# Autodesk Inventor assembly: BoronProbe_5
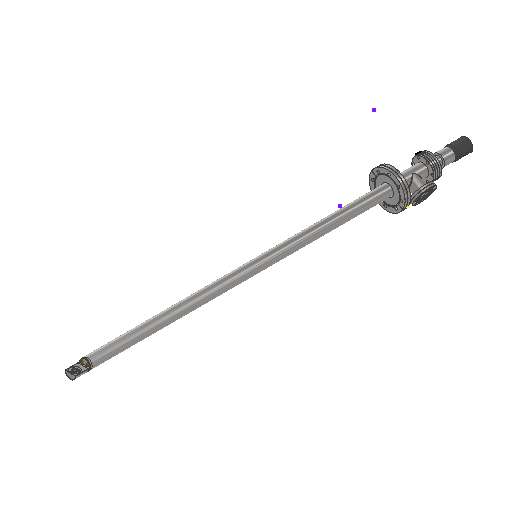
[picture p0: Inventor's stored thumbnail of the model, 512x512]
Saved by Autodesk Inventor 2026.2 (Build 302298000, 298)
## iProperties
Created: 2026-05-08
Part Number: BoronProbe_5
Document SubType Name: Assembly
Designer: zetsu
Author: zetsu
## Documents named in this file (22)
- D:\repos\PIHTI\BoronProbe_5\BoronProbe_5.iam
- D:\repos\PIHTI\BoronProbe_5\parts\B_probehead_5.ipt
- D:\repos\PIHTI\BoronProbe_5\parts\B_holder_sub_5.ipt
- D:\repos\PIHTI\BoronProbe_5\parts\B_pipe_cylinder_5.ipt
- D:\repos\PIHTI\BoronProbe_5\parts\M3x6-BHCS.ipt
- D:\repos\PIHTI\BoronProbe_5\parts\ceramic_bushing_M3-v1.ipt
- D:\repos\PIHTI\BoronProbe_5\parts\ceramic_washer_M4_v1.ipt
- D:\repos\PIHTI\BoronProbe_5\parts\B_shield_5.iam
- D:\repos\PIHTI\BoronProbe_5\parts\ceramic_spacer_d3-13.ipt
- D:\repos\PIHTI\BoronProbe_5\parts\ceramic_2-hole-spacer_d3-13.ipt
- D:\repos\PIHTI\BoronProbe_5\parts\M2-4_screw.ipt
- D:\repos\PIHTI\BoronProbe_5\parts\ICF70TE\ICF70TE.iam
- D:\repos\PIHTI\BoronProbe_5\parts\C25K22A4CU.iam
- D:\repos\PIHTI\BoronProbe_5\parts\substrate.ipt
- D:\repos\PIHTI\BoronProbe_5\parts\M3-nut.ipt
- D:\repos\PIHTI\BoronProbe_5\parts\B_holder_up_5.ipt
- D:\repos\PIHTI\BoronProbe_5\parts\B_probe_pipe_5.ipt
- D:\repos\PIHTI\BoronProbe_5\parts\rotary_transfer_shaft_5.ipt
- D:\repos\PIHTI\BoronProbe_5\parts\Rotary_Feedthrough\Rotary_Feedthrough.iam
- D:\repos\PIHTI\BoronProbe_5\parts\M3x10-BHCS.ipt
- D:\repos\PIHTI\BoronProbe_5\parts\ICF70TE_1.iam
- D:\repos\PIHTI\BoronProbe_5\parts\ICF_114-70.ipt
## Components (39 placed, 20 different names)
1. B_probehead_5:1 — メイト:1, メイト:2, メイト:3, メイト:4, メイト:6, メイト:12, メイト:13, メイト:14, メイト:15, メイト:16, メイト:17, メイト:18, メイト:20, メイト:22, メイト:49, メイト:50, メイト:51, メイト:53, フラッシュ:2, メイト:54, フラッシュ:3, メイト:55, フラッシュ:4
2. B_holder_sub_5:1 — メイト:1, メイト:2, メイト:3, メイト:5, メイト:7, メイト:76, メイト:77, メイト:78, メイト:79, メイト:80, メイト:81, メイト:82, メイト:83, メイト:86
3. Broached Hexagon Socket Button Head Cap Screw - Metric M3 x 0.5 x 6:1 — メイト:4, メイト:5
4. Broached Hexagon Socket Button Head Cap Screw - Metric M3 x 0.5 x 6:2 — メイト:6, メイト:7
5. Broached Hexagon Socket Button Head Cap Screw - Metric M3 x 0.5 x 6:5 — メイト:40, メイト:41
6. ceramic_bushing_M3-v1:1 — メイト:16, メイト:17, メイト:23, メイト:36, メイト:37
7. ceramic_bushing_M3-v1:2 — メイト:14, メイト:15, メイト:19, メイト:40, メイト:41
8. ceramic_bushing_M3-v1:3 — メイト:12, メイト:13, メイト:21, メイト:38, メイト:39
9. ceramic_washer_M4_v1:1 — メイト:20, メイト:21, メイト:43
10. ceramic_washer_M4_v1:2 — メイト:18, メイト:19, メイト:42
11. ceramic_washer_M4_v1:3 — メイト:22, メイト:23, メイト:44
12. Broached Hexagon Socket Button Head Cap Screw - Metric M3 x 0.5 x 6:6 — メイト:38, メイト:39
13. Broached Hexagon Socket Button Head Cap Screw - Metric M3 x 0.5 x 6:7 — メイト:36, メイト:37
14. B_pipe_cylinder_5:1 — メイト:42, メイト:43, メイト:44, メイト:93, メイト:94
15. B_shield_5:1 [sub-assembly] — メイト:49, メイト:50, メイト:51, メイト:56, メイト:57, メイト:58, メイト:59
16. ceramic_spacer_d3-13:1 — メイト:53, フラッシュ:2
17. ceramic_spacer_d3-13:2 — メイト:54, フラッシュ:3
18. ceramic_2-hole-spacer_d3-13:1 — メイト:55, フラッシュ:4
19. M2-4_screw:1 — メイト:56, メイト:57
20. M2-4_screw:2 — メイト:58, メイト:59
21. C25K22A4CU:1 [sub-assembly]
22. substrate:1 — メイト:76, メイト:77, メイト:84
23. JIS B 1181 Style 1 - Metric A M3:1 — メイト:78, メイト:79
24. JIS B 1181 Style 1 - Metric A M3:2 — メイト:82, メイト:83
25. JIS B 1181 Style 1 - Metric A M3:3 — メイト:80, メイト:81, メイト:85
26. B_holder_up_5:1 — メイト:84, メイト:85, メイト:86, メイト:87, メイト:88, メイト:89, メイト:90, メイト:91, メイト:92
27. Broached Hexagon Socket Button Head Cap Screw - Metric M3 x 0.5 x 6:8 — メイト:87, メイト:88
28. Broached Hexagon Socket Button Head Cap Screw - Metric M3 x 0.5 x 6:9 — メイト:89, メイト:90
29. Broached Hexagon Socket Button Head Cap Screw - Metric M3 x 0.5 x 6:10 — メイト:91, メイト:92
30. B_probe_pipe_5:1 — メイト:93, メイト:94, メイト:95, メイト:96, メイト:99, メイト:100, メイト:101, メイト:102, メイト:103, メイト:104, メイト:105, メイト:106
31. rotary_transfer_shaft_5:1 — メイト:95, メイト:96, メイト:97, メイト:98
32. Rotary_Feedthrough:1 [sub-assembly] — メイト:97, メイト:98, メイト:107, メイト:108, メイト:109, メイト:110, メイト:111, メイト:112
33. Broached Hexagon Socket Button Head Cap Screw - Metric M3 x 0.5 x 6:11 — メイト:99, メイト:100
34. Broached Hexagon Socket Button Head Cap Screw - Metric M3 x 0.5 x 6:12 — メイト:101, メイト:102
35. Broached Hexagon Socket Button Head Cap Screw - Metric M3 x 0.5 x 6:13 — メイト:103, メイト:104
36. Broached Hexagon Socket Button Head Cap Screw - Metric M3 x 0.5 x 6:14 — メイト:105, メイト:106
37. ICF70TE_1:1 [sub-assembly] — メイト:107, メイト:108, メイト:109
38. ICF70TE:2 [sub-assembly] — メイト:110, メイト:111, メイト:112, メイト:113, メイト:114, メイト:115
39. ICF_114-70:1 — メイト:113, メイト:114, メイト:115
## Relationships (81: Mate 78, Flush 3)
- メイト:1 [Mate]: B_probehead_5:1 ↔ B_holder_sub_5:1
- メイト:2 [Mate]: B_probehead_5:1 ↔ B_holder_sub_5:1
- メイト:3 [Mate]: B_probehead_5:1 ↔ B_holder_sub_5:1
- メイト:4 [Mate]: B_probehead_5:1 ↔ Broached Hexagon Socket Button Head Cap Screw - Metric M3 x 0.5 x 6:1
- メイト:5 [Mate]: B_holder_sub_5:1 ↔ Broached Hexagon Socket Button Head Cap Screw - Metric M3 x 0.5 x 6:1
- メイト:6 [Mate]: B_probehead_5:1 ↔ Broached Hexagon Socket Button Head Cap Screw - Metric M3 x 0.5 x 6:2
- メイト:7 [Mate]: B_holder_sub_5:1 ↔ Broached Hexagon Socket Button Head Cap Screw - Metric M3 x 0.5 x 6:2
- メイト:12 [Mate]: B_probehead_5:1 ↔ ceramic_bushing_M3-v1:3
- メイト:13 [Mate]: B_probehead_5:1 ↔ ceramic_bushing_M3-v1:3
- メイト:14 [Mate]: B_probehead_5:1 ↔ ceramic_bushing_M3-v1:2
- メイト:15 [Mate]: B_probehead_5:1 ↔ ceramic_bushing_M3-v1:2
- メイト:16 [Mate]: B_probehead_5:1 ↔ ceramic_bushing_M3-v1:1
- メイト:17 [Mate]: B_probehead_5:1 ↔ ceramic_bushing_M3-v1:1
- メイト:18 [Mate]: B_probehead_5:1 ↔ ceramic_washer_M4_v1:2
- メイト:19 [Mate]: ceramic_bushing_M3-v1:2 ↔ ceramic_washer_M4_v1:2
- メイト:20 [Mate]: B_probehead_5:1 ↔ ceramic_washer_M4_v1:1
- メイト:21 [Mate]: ceramic_bushing_M3-v1:3 ↔ ceramic_washer_M4_v1:1
- メイト:22 [Mate]: B_probehead_5:1 ↔ ceramic_washer_M4_v1:3
- メイト:23 [Mate]: ceramic_bushing_M3-v1:1 ↔ ceramic_washer_M4_v1:3
- メイト:36 [Mate]: ceramic_bushing_M3-v1:1 ↔ Broached Hexagon Socket Button Head Cap Screw - Metric M3 x 0.5 x 6:7
- メイト:37 [Mate]: ceramic_bushing_M3-v1:1 ↔ Broached Hexagon Socket Button Head Cap Screw - Metric M3 x 0.5 x 6:7
- メイト:38 [Mate]: ceramic_bushing_M3-v1:3 ↔ Broached Hexagon Socket Button Head Cap Screw - Metric M3 x 0.5 x 6:6
- メイト:39 [Mate]: ceramic_bushing_M3-v1:3 ↔ Broached Hexagon Socket Button Head Cap Screw - Metric M3 x 0.5 x 6:6
- メイト:40 [Mate]: Broached Hexagon Socket Button Head Cap Screw - Metric M3 x 0.5 x 6:5 ↔ ceramic_bushing_M3-v1:2
- メイト:41 [Mate]: Broached Hexagon Socket Button Head Cap Screw - Metric M3 x 0.5 x 6:5 ↔ ceramic_bushing_M3-v1:2
- メイト:42 [Mate]: ceramic_washer_M4_v1:2 ↔ B_pipe_cylinder_5:1
- メイト:43 [Mate]: ceramic_washer_M4_v1:1 ↔ B_pipe_cylinder_5:1
- メイト:44 [Mate]: ceramic_washer_M4_v1:3 ↔ B_pipe_cylinder_5:1
- メイト:49 [Mate]: B_probehead_5:1 ↔ B_shield_5:1
- メイト:50 [Mate]: B_probehead_5:1 ↔ B_shield_5:1
- メイト:51 [Mate]: B_probehead_5:1 ↔ B_shield_5:1
- メイト:53 [Mate]: B_probehead_5:1 ↔ ceramic_spacer_d3-13:1
- フラッシュ:2 [Flush]: B_probehead_5:1 ↔ ceramic_spacer_d3-13:1
- メイト:54 [Mate]: B_probehead_5:1 ↔ ceramic_spacer_d3-13:2
- フラッシュ:3 [Flush]: B_probehead_5:1 ↔ ceramic_spacer_d3-13:2
- メイト:55 [Mate]: B_probehead_5:1 ↔ ceramic_2-hole-spacer_d3-13:1
- フラッシュ:4 [Flush]: B_probehead_5:1 ↔ ceramic_2-hole-spacer_d3-13:1
- メイト:56 [Mate]: B_shield_5:1 ↔ M2-4_screw:1
- メイト:57 [Mate]: B_shield_5:1 ↔ M2-4_screw:1
- メイト:58 [Mate]: B_shield_5:1 ↔ M2-4_screw:2
- メイト:59 [Mate]: B_shield_5:1 ↔ M2-4_screw:2
- メイト:76 [Mate]: B_holder_sub_5:1 ↔ substrate:1
- メイト:77 [Mate]: B_holder_sub_5:1 ↔ substrate:1
- メイト:78 [Mate]: B_holder_sub_5:1 ↔ JIS B 1181 Style 1 - Metric A M3:1
- メイト:79 [Mate]: B_holder_sub_5:1 ↔ JIS B 1181 Style 1 - Metric A M3:1
- メイト:80 [Mate]: B_holder_sub_5:1 ↔ JIS B 1181 Style 1 - Metric A M3:3
- メイト:81 [Mate]: B_holder_sub_5:1 ↔ JIS B 1181 Style 1 - Metric A M3:3
- メイト:82 [Mate]: B_holder_sub_5:1 ↔ JIS B 1181 Style 1 - Metric A M3:2
- メイト:83 [Mate]: B_holder_sub_5:1 ↔ JIS B 1181 Style 1 - Metric A M3:2
- メイト:84 [Mate]: substrate:1 ↔ B_holder_up_5:1
- メイト:85 [Mate]: JIS B 1181 Style 1 - Metric A M3:3 ↔ B_holder_up_5:1
- メイト:86 [Mate]: B_holder_sub_5:1 ↔ B_holder_up_5:1
- メイト:87 [Mate]: B_holder_up_5:1 ↔ Broached Hexagon Socket Button Head Cap Screw - Metric M3 x 0.5 x 6:8
- メイト:88 [Mate]: B_holder_up_5:1 ↔ Broached Hexagon Socket Button Head Cap Screw - Metric M3 x 0.5 x 6:8
- メイト:89 [Mate]: B_holder_up_5:1 ↔ Broached Hexagon Socket Button Head Cap Screw - Metric M3 x 0.5 x 6:9
- メイト:90 [Mate]: B_holder_up_5:1 ↔ Broached Hexagon Socket Button Head Cap Screw - Metric M3 x 0.5 x 6:9
- メイト:91 [Mate]: B_holder_up_5:1 ↔ Broached Hexagon Socket Button Head Cap Screw - Metric M3 x 0.5 x 6:10
- メイト:92 [Mate]: B_holder_up_5:1 ↔ Broached Hexagon Socket Button Head Cap Screw - Metric M3 x 0.5 x 6:10
- メイト:93 [Mate]: B_pipe_cylinder_5:1 ↔ B_probe_pipe_5:1
- メイト:94 [Mate]: B_pipe_cylinder_5:1 ↔ B_probe_pipe_5:1
- メイト:95 [Mate]: B_probe_pipe_5:1 ↔ rotary_transfer_shaft_5:1
- メイト:96 [Mate]: B_probe_pipe_5:1 ↔ rotary_transfer_shaft_5:1
- メイト:97 [Mate]: rotary_transfer_shaft_5:1 ↔ Rotary_Feedthrough:1
- メイト:98 [Mate]: rotary_transfer_shaft_5:1 ↔ Rotary_Feedthrough:1
- メイト:99 [Mate]: B_probe_pipe_5:1 ↔ Broached Hexagon Socket Button Head Cap Screw - Metric M3 x 0.5 x 6:11
- メイト:100 [Mate]: B_probe_pipe_5:1 ↔ Broached Hexagon Socket Button Head Cap Screw - Metric M3 x 0.5 x 6:11
- メイト:101 [Mate]: B_probe_pipe_5:1 ↔ Broached Hexagon Socket Button Head Cap Screw - Metric M3 x 0.5 x 6:12
- メイト:102 [Mate]: B_probe_pipe_5:1 ↔ Broached Hexagon Socket Button Head Cap Screw - Metric M3 x 0.5 x 6:12
- メイト:103 [Mate]: B_probe_pipe_5:1 ↔ Broached Hexagon Socket Button Head Cap Screw - Metric M3 x 0.5 x 6:13
- メイト:104 [Mate]: B_probe_pipe_5:1 ↔ Broached Hexagon Socket Button Head Cap Screw - Metric M3 x 0.5 x 6:13
- メイト:105 [Mate]: B_probe_pipe_5:1 ↔ Broached Hexagon Socket Button Head Cap Screw - Metric M3 x 0.5 x 6:14
- メイト:106 [Mate]: B_probe_pipe_5:1 ↔ Broached Hexagon Socket Button Head Cap Screw - Metric M3 x 0.5 x 6:14
- メイト:107 [Mate]: Rotary_Feedthrough:1 ↔ ICF70TE_1:1
- メイト:108 [Mate]: Rotary_Feedthrough:1 ↔ ICF70TE_1:1
- メイト:109 [Mate]: Rotary_Feedthrough:1 ↔ ICF70TE_1:1
- メイト:110 [Mate]: Rotary_Feedthrough:1 ↔ ICF70TE:2
- メイト:111 [Mate]: Rotary_Feedthrough:1 ↔ ICF70TE:2
- メイト:112 [Mate]: Rotary_Feedthrough:1 ↔ ICF70TE:2
- メイト:113 [Mate]: ICF70TE:2 ↔ ICF_114-70:1
- メイト:114 [Mate]: ICF70TE:2 ↔ ICF_114-70:1
- メイト:115 [Mate]: ICF70TE:2 ↔ ICF_114-70:1
